# Autodesk Inventor assembly: Binary Clock
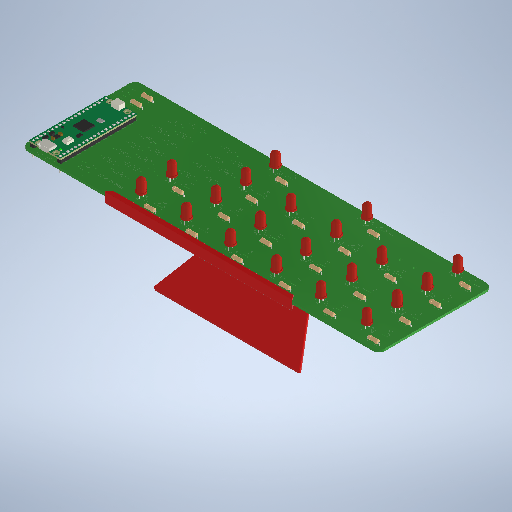
[picture p0: Inventor's stored thumbnail of the model, 512x512]
Saved by Autodesk Inventor 2025.3 (Build 293356000, 356)
## iProperties
Company: Kicad
Created: 2025-11-09
Part Number: Binary Clock
Description: KiCad electronic assembly
Document SubType Name: Assembly
Designer: User
Authority: Unknown
Sending System: KiCad to STEP converter
Preprocessor: Open CASCADE STEP processor 7.9
Title: Binary Clock.step
Author: Pcbnew
## Documents named in this file (7)
- C:\Users\User\Documents\KiCad\Binary Clock\Binary Clock\Binary Clock\Binary Clock\Binary Clock.iam
- C:\Users\User\Documents\KiCad\Binary Clock\Binary Clock\Binary Clock\Binary Clock\LED_D5.0mm.ipt
- C:\Users\User\Documents\KiCad\Binary Clock\Binary Clock\Binary Clock\Binary Clock\R_Axial_DIN0207_L6.3mm_D2.5mm_P7.62mm_Horizontal.ipt
- C:\Users\User\Documents\KiCad\Binary Clock\Binary Clock\Binary Clock\Binary Clock\RaspberryPi_Pico_H.iam
- C:\Users\User\Documents\KiCad\Binary Clock\Binary Clock\Binary Clock\Binary Clock\Binary Clock_silkscreen.ipt
- C:\Users\User\Documents\KiCad\Binary Clock\Binary Clock\Binary Clock\Binary Clock\Binary Clock_PCB.ipt
- C:\Users\User\3D\PC Case\Part14.ipt
## Components (46 placed, 46 different names)
1. 1
2. 2
3. 3
4. 4
5. 5
6. 6
7. 7
8. 8
9. 9
10. 10
11. 11
12. 12
13. 13
14. 14
15. 15
16. 16
17. 17
18. 18
19. 19
20. 20
21. 21
22. 22
23. 23
24. 24
25. 25
26. 26
27. 27
28. 28
29. 29
30. 30
31. 31
32. 32
33. 33
34. 34
35. 35
36. 36
37. 39 [sub-assembly]
38. 40
39. 41
40. 42
41. 43
42. 44
43. 45
44. 46
45. 47 — Flush:1
46. Part14:1 — Flush:1
## Relationships (1: Flush 1)
- Flush:1: 47 ↔ Part14:1
